# Autodesk Inventor assembly: Assembly
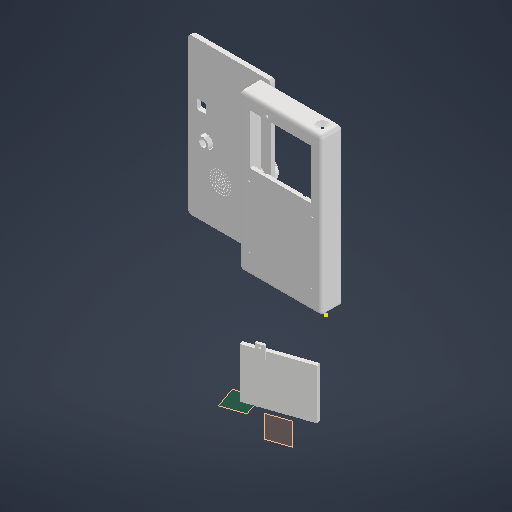
[picture p0: Inventor's stored thumbnail of the model, 512x512]
Saved by Autodesk Inventor 2027 (Build 310192000, 192)
## iProperties
Created: 2026-03-08
Part Number: Assembly
Document SubType Name: Assembly
Designer: kjedr
Author: kjedr
## Documents named in this file (6)
- D:\LAST SEMESTER\ECE445-UIUC-Heterodyne\Chassis\Assembly.iam
- D:\LAST SEMESTER\ECE445-UIUC-Heterodyne\Chassis\Top_Shell.ipt
- D:\LAST SEMESTER\ECE445-UIUC-Heterodyne\Chassis\Bottom_Shell.ipt
- D:\LAST SEMESTER\ECE445-UIUC-Heterodyne\Chassis\Dial.ipt
- D:\LAST SEMESTER\ECE445-UIUC-Heterodyne\Chassis\batteryFlap.ipt
- D:\LAST SEMESTER\ECE445-UIUC-Heterodyne\Chassis\freqDial1.ipt
## Components (5 placed, 5 different names)
1. Top_Shell:1 — Insert:1, Insert:2
2. Bottom_Shell:1
3. Dial:2 — Insert:1
4. batteryFlap:1
5. freqDial1:1 — Insert:2
## Relationships (2: Insert 2)
- Insert:1: Top_Shell:1 ↔ Dial:2
- Insert:2: Top_Shell:1 ↔ freqDial1:1
